# Autodesk Inventor assembly: BOX_PART
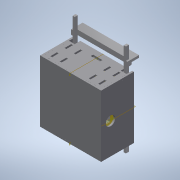
[picture p0: Inventor's stored thumbnail of the model, 180x180]
Saved by Autodesk Inventor 2020 (Build 240168000, 168)
## iProperties
Created: 2019-12-17
Part Number: BOX_PART
Document SubType Name: Assembly
Designer: fabfarm
Author: fabfarm
## Documents named in this file (6)
- D:\fablab\sawbench\BOX_PART.iam
- D:\fablab\sawbench\Side_one.ipt
- D:\fablab\sawbench\Side_two.ipt
- D:\fablab\sawbench\TableSaw_Bench3.ipt
- D:\fablab\sawbench\bottom-case.ipt
- D:\fablab\sawbench\open_case.ipt
## Components (6 placed, 5 different names)
1. Side_one:1 — Flush:4, Flush:5, Symmetry:1, Placage:11, Placage:12
2. Side_two:1 — Mate:10, Flush:4, Flush:7, Symmetry:2, Placage:12, Affleurement:12
3. TableSaw_Bench3:1 — Flush:6, Flush:9, Affleurement:13, Placage:15, Affleurement:14
4. Side_one:2 — Flush:6, Flush:7, Flush:8, Flush:10, Symmetry:1, Placage:13, Affleurement:11, Affleurement:12, Placage:14
5. bottom-case:1 — Mate:10, Flush:5, Flush:8, Placage:11, Placage:13, Affleurement:11
6. open_case:1 — Flush:9, Flush:10, Symmetry:2, Placage:14
## Relationships (19: Flush 11, Mate 6, Symmetry 2)
- Mate:10: Side_two:1 ↔ bottom-case:1
- Flush:4: Side_one:1 ↔ Side_two:1
- Flush:5: Side_one:1 ↔ bottom-case:1
- Flush:6: TableSaw_Bench3:1 ↔ Side_one:2
- Flush:7: Side_two:1 ↔ Side_one:2
- Flush:8: Side_one:2 ↔ bottom-case:1
- Flush:9: TableSaw_Bench3:1 ↔ open_case:1
- Flush:10: Side_one:2 ↔ open_case:1
- Symmetry:1: Side_one:1 ↔ Side_one:2
- Symmetry:2: Side_two:1 ↔ open_case:1
- Placage:11 [Mate]: Side_one:1 ↔ bottom-case:1
- Placage:12 [Mate]: Side_one:1 ↔ Side_two:1
- Placage:13 [Mate]: Side_one:2 ↔ bottom-case:1
- Affleurement:11 [Flush]: Side_one:2 ↔ bottom-case:1
- Affleurement:12 [Flush]: Side_two:1 ↔ Side_one:2
- Placage:14 [Mate]: Side_one:2 ↔ open_case:1
- Affleurement:13 [Flush]: TableSaw_Bench3:1
- Placage:15 [Mate]: TableSaw_Bench3:1
- Affleurement:14 [Flush]: TableSaw_Bench3:1
